# Autodesk Inventor assembly: Maccaronikanone
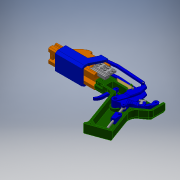
[picture p0: Inventor's stored thumbnail of the model, 180x180]
Saved by Autodesk Inventor 2019 (Build 230136000, 136)
## iProperties
Created: 2021-03-07
Part Number: Maccaronikanone
Document SubType Name: Assembly
Designer: Lukas
Author: Lukas
## Documents named in this file (19)
- \\192.168.1.200\Storragepool\Datastorrage\CAD\Inventor 2019\Maccaronikanone\Maccaronikanone.iam
- \\192.168.1.200\Storragepool\Datastorrage\CAD\Inventor 2019\Maccaronikanone\Griff_rechts.ipt
- \\192.168.1.200\Storragepool\Datastorrage\CAD\Inventor 2019\Maccaronikanone\Hammer.ipt
- \\192.168.1.200\Storragepool\Datastorrage\CAD\Inventor 2019\Maccaronikanone\Hammer_Knautschzone.ipt
- \\192.168.1.200\Storragepool\Datastorrage\CAD\Inventor 2019\Maccaronikanone\Fangklinke.ipt
- \\192.168.1.200\Storragepool\Datastorrage\CAD\Inventor 2019\Maccaronikanone\Abzugstange.ipt
- \\192.168.1.200\Storragepool\Datastorrage\CAD\Inventor 2019\Maccaronikanone\Abzug.ipt
- \\192.168.1.200\Storragepool\Datastorrage\CAD\Inventor 2019\Maccaronikanone\Ladelasche_links.ipt
- \\192.168.1.200\Storragepool\Datastorrage\CAD\Inventor 2019\Maccaronikanone\Ladelasche_rechts.ipt
- \\192.168.1.200\Storragepool\Datastorrage\CAD\Inventor 2019\Maccaronikanone\Griff_links.ipt
- \\192.168.1.200\Storragepool\Datastorrage\CAD\Inventor 2019\Maccaronikanone\Ladelasche_Schraube.ipt
- \\192.168.1.200\Storragepool\Datastorrage\CAD\Inventor 2019\Maccaronikanone\Federgelenkblock.ipt
- \\192.168.1.200\Storragepool\Datastorrage\CAD\Inventor 2019\Maccaronikanone\Federstange.ipt
- \\192.168.1.200\Storragepool\Datastorrage\CAD\Inventor 2019\Maccaronikanone\Magazinhalter und Laderampe.ipt
- \\192.168.1.200\Storragepool\Datastorrage\CAD\Inventor 2019\Maccaronikanone\Ladeschlitten.ipt
- \\192.168.1.200\Storragepool\Datastorrage\CAD\Inventor 2019\Maccaronikanone\Ladebügel.ipt
- \\192.168.1.200\Storragepool\Datastorrage\CAD\Inventor 2019\Maccaronikanone\Maccaroni.ipt
- \\192.168.1.200\Storragepool\Datastorrage\CAD\Inventor 2019\Maccaronikanone\Montageplatte_L.ipt
- \\192.168.1.200\Storragepool\Datastorrage\CAD\Inventor 2019\Maccaronikanone\Montageplatte_R.ipt
## Components (20 placed, 18 different names)
1. Griff_rechts:1 — Flush:1, Flush:2, Flush:3, Mate:1, Mate:2, Mate:8, Mate:9, Mate:15, Mate:24, Mate:27, Mate:28, Flush:7, Mate:31, Mate:34, Mate:37, Flush:10, Mate:38, Flush:11, Flush:12, Angle:5, Mate:46, Flush:15, Mate:53, Mate:54
2. Griff_links:1 — Flush:7, Mate:31, Flush:10, Flush:14, Mate:51, Mate:52
3. Hammer:1 — Mate:1, Mate:2, Mate:3, Mate:4, Flush:4, Mate:29, Mate:30, Mate:35, Tangent:1, Tangent:2
4. Hammer_Knautschzone:1 — Mate:3, Mate:4, Flush:4
5. Fangklinke:1 — Mate:8, Mate:9, Mate:12, Mate:25
6. Abzugstange:1 — Mate:12, Mate:25, Mate:26
7. Abzug:1 — Mate:15, Mate:24, Mate:26
8. Ladelasche_links:1 — Mate:29, Mate:30, Flush:5, Angle:5
9. Ladelasche_rechts:1 — Mate:27, Mate:28, Flush:5, Mate:32, Angle:3, Mate:33, Flush:9
10. Ladelasche_Schraube:1 — Mate:32, Angle:3, Angle:4, Mate:42, Mate:50, Flush:13
11. Ladelasche_Schraube:2 — Mate:33, Flush:9, Angle:4, Tangent:2
12. Federgelenkblock:1 — Mate:34, Mate:36, Mate:37
13. Federstange:1 — Mate:35, Tangent:1, Mate:36
14. Magazinhalter und Laderampe:1 — Mate:38, Flush:11, Flush:12, Mate:40, Mate:41
15. Ladeschlitten:1 — Mate:40, Mate:41, Mate:44, Mate:47, Mate:48, Mate:49
16. Ladebügel:1 — Mate:42, Mate:44, Mate:47, Flush:13
17. Ladebügel:2 — Mate:48, Mate:49, Mate:50
18. Maccaroni:1 — Mate:46
19. Montageplatte_L:1 — Flush:14, Mate:51, Mate:52
20. Montageplatte_R:1 — Flush:15, Mate:53, Mate:54
## Relationships (54: Mate 36, Flush 13, Angle 3, Tangent 2)
- Flush:1: Griff_rechts:1
- Flush:2: Griff_rechts:1
- Flush:3 (15.5 mm): Griff_rechts:1
- Mate:1: Griff_rechts:1 ↔ Hammer:1
- Mate:2 (2 mm): Griff_rechts:1 ↔ Hammer:1
- Mate:3: Hammer:1 ↔ Hammer_Knautschzone:1
- Mate:4: Hammer:1 ↔ Hammer_Knautschzone:1
- Flush:4: Hammer:1 ↔ Hammer_Knautschzone:1
- Mate:8: Griff_rechts:1 ↔ Fangklinke:1
- Mate:9: Griff_rechts:1 ↔ Fangklinke:1
- Mate:12: Fangklinke:1 ↔ Abzugstange:1
- Mate:15 (0.2 mm): Griff_rechts:1 ↔ Abzug:1
- Mate:24: Griff_rechts:1 ↔ Abzug:1
- Mate:25 (0.1 mm): Fangklinke:1 ↔ Abzugstange:1
- Mate:26: Abzugstange:1 ↔ Abzug:1
- Mate:27 (0.1 mm): Griff_rechts:1 ↔ Ladelasche_rechts:1
- Mate:28: Griff_rechts:1 ↔ Ladelasche_rechts:1
- Mate:29 (0.1 mm): Hammer:1 ↔ Ladelasche_links:1
- Mate:30: Hammer:1 ↔ Ladelasche_links:1
- Flush:5: Ladelasche_links:1 ↔ Ladelasche_rechts:1
- Flush:7: Griff_rechts:1 ↔ Griff_links:1
- Mate:31: Griff_rechts:1 ↔ Griff_links:1
- Mate:32: Ladelasche_rechts:1 ↔ Ladelasche_Schraube:1
- Angle:3 (0 deg): Ladelasche_rechts:1 ↔ Ladelasche_Schraube:1
- Mate:33: Ladelasche_rechts:1 ↔ Ladelasche_Schraube:2
- Flush:9 (3.6 mm): Ladelasche_rechts:1 ↔ Ladelasche_Schraube:2
- Angle:4 (0 deg): Ladelasche_Schraube:1 ↔ Ladelasche_Schraube:2
- Mate:34: Griff_rechts:1 ↔ Federgelenkblock:1
- Mate:35: Hammer:1 ↔ Federstange:1
- Tangent:1: Hammer:1 ↔ Federstange:1
- Mate:36: Federgelenkblock:1 ↔ Federstange:1
- Mate:37: Griff_rechts:1 ↔ Federgelenkblock:1
- Flush:10: Griff_rechts:1 ↔ Griff_links:1
- Mate:38 (0.1 mm): Griff_rechts:1 ↔ Magazinhalter und Laderampe:1
- Flush:11: Griff_rechts:1 ↔ Magazinhalter und Laderampe:1
- Flush:12: Griff_rechts:1 ↔ Magazinhalter und Laderampe:1
- Mate:40 (0.3 mm): Magazinhalter und Laderampe:1 ↔ Ladeschlitten:1
- Mate:41 (0.3 mm): Magazinhalter und Laderampe:1 ↔ Ladeschlitten:1
- Mate:42: Ladelasche_Schraube:1 ↔ Ladebügel:1
- Mate:44: Ladeschlitten:1 ↔ Ladebügel:1
- Tangent:2: Hammer:1 ↔ Ladelasche_Schraube:2
- Angle:5 (0 deg): Griff_rechts:1 ↔ Ladelasche_links:1
- Mate:46: Griff_rechts:1 ↔ Maccaroni:1
- Mate:47 (0.1 mm): Ladeschlitten:1 ↔ Ladebügel:1
- Mate:48: Ladeschlitten:1 ↔ Ladebügel:2
- Mate:49 (0.1 mm): Ladeschlitten:1 ↔ Ladebügel:2
- Mate:50: Ladelasche_Schraube:1 ↔ Ladebügel:2
- Flush:13: Ladelasche_Schraube:1 ↔ Ladebügel:1
- Flush:14: Griff_links:1 ↔ Montageplatte_L:1
- Mate:51 (0.3 mm): Griff_links:1 ↔ Montageplatte_L:1
- Mate:52 (0.2 mm): Griff_links:1 ↔ Montageplatte_L:1
- Flush:15: Griff_rechts:1 ↔ Montageplatte_R:1
- Mate:53 (0.3 mm): Griff_rechts:1 ↔ Montageplatte_R:1
- Mate:54 (0.2 mm): Griff_rechts:1 ↔ Montageplatte_R:1
